# Autodesk Inventor assembly: chwytak
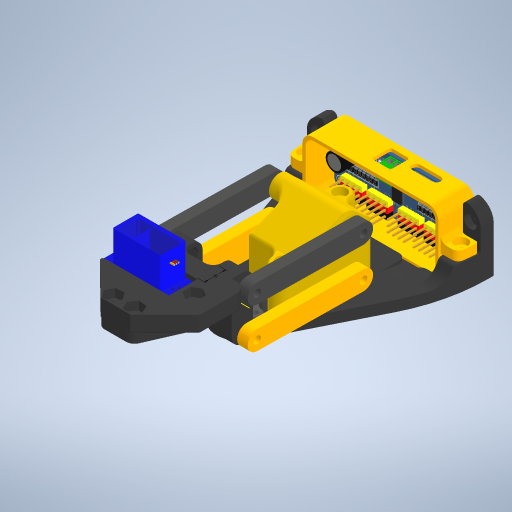
[picture p0: Inventor's stored thumbnail of the model, 512x512]
Saved by Autodesk Inventor 2023 (Build 270158000, 158)
## iProperties
Created: 2024-05-12
Part Number: chwytak
Document SubType Name: Assembly
Designer: kamil
Author: kamil
## Documents named in this file (12)
- C:\Users\kamil\Documents\PROJECTS - repos\ModBot---Projekt-Zespolowy\mechanics\modul_chwytaka\chwytak.iam
- C:\Users\kamil\Documents\PROJECTS - repos\ModBot---Projekt-Zespolowy\mechanics\modul_chwytaka\belka.ipt
- C:\Users\kamil\Documents\PROJECTS - repos\ModBot---Projekt-Zespolowy\mechanics\modul_chwytaka\Towerpro Micro Servo 9g.ipt
- C:\Users\kamil\Documents\PROJECTS - repos\ModBot---Projekt-Zespolowy\mechanics\modul_chwytaka\A1.ipt
- C:\Users\kamil\Documents\PROJECTS - repos\ModBot---Projekt-Zespolowy\mechanics\modul_chwytaka\uchwyt_serwa.ipt
- C:\Users\kamil\Documents\PROJECTS - repos\ModBot---Projekt-Zespolowy\mechanics\modul_chwytaka\belka_2.ipt
- C:\Users\kamil\Documents\PROJECTS - repos\ModBot---Projekt-Zespolowy\mechanics\modul_chwytaka\uchwyt_gorny.ipt
- C:\Users\kamil\Documents\PROJECTS - repos\ModBot---Projekt-Zespolowy\mechanics\STEP\pca9685.ipt
- C:\Users\kamil\Documents\PROJECTS - repos\ModBot---Projekt-Zespolowy\mechanics\chwytak_mocowanie.ipt
- C:\Users\kamil\Documents\PROJECTS - repos\ModBot---Projekt-Zespolowy\mechanics\STEP\Pololu Ball Caster with 3_8_ Metal Ball.ipt
- C:\Users\kamil\Documents\PROJECTS - repos\ModBot---Projekt-Zespolowy\mechanics\pca_obudowa.iam
- C:\Users\kamil\Documents\PROJECTS - repos\ModBot---Projekt-Zespolowy\mechanics\modul_chwytaka\chwytak_montaz.ipt
## Components (15 placed, 11 different names)
1. belka:1 — Zestawiające:4, Zestawiające:5, Kątowe:1, Zestawiające:12, Równoległe:3, Równoległe:6, Zestawiające:46
2. Towerpro Micro Servo 9g:1 — Zestawiające:1, Zestawiające:2, Równoległe:1, Zestawiające:3, Zestawiające:6, Zestawiające:7, Zestawiające:8, Zestawiające:9
3. A1:1 — Zestawiające:2, Zestawiające:3, Zestawiające:4, Zestawiające:5, Kątowe:1
4. uchwyt_serwa:1 — Zestawiające:7, Zestawiające:8, Zestawiające:9, Zestawiające:10, Zestawiające:11, Zestawiające:13, Zestawiające:14, Zestawiające:37, Zestawiające:40
5. belka_2:1 — Zestawiające:10, Zestawiające:11, Zestawiające:12, Równoległe:2, Kątowe:2
6. uchwyt_gorny:1 — Zestawiające:13, Zestawiające:14, Zestawiające:38, Zestawiające:39
7. belka_2:2 — Równoległe:2, Kątowe:2, Równoległe:4, Zestawiające:39
8. belka_2:3 — Równoległe:3, Równoległe:4, Zestawiające:38, Zestawiające:47, Zestawiające:48
9. chwytak_mocowanie:1 — Zestawiające:35, Zestawiające:36, Zestawiające:37, Równoległe:5, Równoległe:6, Zestawiające:40, Zestawiające:41, Zestawiające:42, Zestawiające:43, Zestawiające:44, Równoległe:7, Równoległe:8, Zestawiające:45, Równoległe:9
10. Pololu Ball Caster with 3_8_ Metal Ball:1 — Zestawiające:41, Zestawiające:42, Zestawiające:43, Zestawiające:44
11. pca9685:1 — Zestawiające:35, Zestawiające:36, Równoległe:5
12. pca_obudowa:1 [sub-assembly] — Równoległe:7, Równoległe:8, Zestawiające:45, Równoległe:9, Zestawiające:52, Zestawiające:53, Zestawiające:54
13. chwytak_montaz:1 — Zestawiające:46, Zestawiające:47, Zestawiające:48, Zestawiające:49, Kątowe:3, Zestawiające:50, Zestawiające:51
14. Towerpro Micro Servo 9g:2 — Zestawiające:49, Kątowe:3, Zestawiające:50, Zestawiające:51
15. pca9685:2 — Zestawiające:52, Zestawiające:53, Zestawiające:54
## Relationships (46: Mate 34, Flush 9, Angle 3)
- Zestawiające:1 [Mate]: Towerpro Micro Servo 9g:1
- Zestawiające:2 [Mate]: Towerpro Micro Servo 9g:1 ↔ A1:1
- Równoległe:1 [Flush]: Towerpro Micro Servo 9g:1
- Zestawiające:3 [Mate]: Towerpro Micro Servo 9g:1 ↔ A1:1
- Zestawiające:4 [Mate]: belka:1 ↔ A1:1
- Zestawiające:5 [Mate]: belka:1 ↔ A1:1
- Kątowe:1 [Angle] (180 deg): belka:1 ↔ A1:1
- Zestawiające:6 [Mate]: Towerpro Micro Servo 9g:1
- Zestawiające:7 [Mate]: Towerpro Micro Servo 9g:1 ↔ uchwyt_serwa:1
- Zestawiające:8 [Mate] (0.5 mm): Towerpro Micro Servo 9g:1 ↔ uchwyt_serwa:1
- Zestawiające:9 [Mate]: Towerpro Micro Servo 9g:1 ↔ uchwyt_serwa:1
- Zestawiające:10 [Mate] (2 mm): uchwyt_serwa:1 ↔ belka_2:1
- Zestawiające:11 [Mate]: uchwyt_serwa:1 ↔ belka_2:1
- Zestawiające:12 [Mate]: belka:1 ↔ belka_2:1
- Zestawiające:13 [Mate]: uchwyt_serwa:1 ↔ uchwyt_gorny:1
- Zestawiające:14 [Mate]: uchwyt_serwa:1 ↔ uchwyt_gorny:1
- Równoległe:2 [Flush]: belka_2:1 ↔ belka_2:2
- Kątowe:2 [Angle] (180 deg): belka_2:1 ↔ belka_2:2
- Równoległe:3 [Flush]: belka:1 ↔ belka_2:3
- Równoległe:4 [Flush]: belka_2:2 ↔ belka_2:3
- Zestawiające:35 [Mate] (2 mm): chwytak_mocowanie:1 ↔ pca9685:1
- Zestawiające:36 [Mate] (2 mm): chwytak_mocowanie:1 ↔ pca9685:1
- Zestawiające:37 [Mate]: uchwyt_serwa:1 ↔ chwytak_mocowanie:1
- Równoległe:5 [Flush] (-11 mm): chwytak_mocowanie:1 ↔ pca9685:1
- Zestawiające:38 [Mate]: uchwyt_gorny:1 ↔ belka_2:3
- Zestawiające:39 [Mate]: uchwyt_gorny:1 ↔ belka_2:2
- Równoległe:6 [Flush] (17.75 mm): belka:1 ↔ chwytak_mocowanie:1
- Zestawiające:40 [Mate] (25 mm): uchwyt_serwa:1 ↔ chwytak_mocowanie:1
- Zestawiające:41 [Mate] (-7 mm): chwytak_mocowanie:1 ↔ Pololu Ball Caster with 3_8_ Metal Ball:1
- Zestawiające:42 [Mate] (-41 mm): chwytak_mocowanie:1 ↔ Pololu Ball Caster with 3_8_ Metal Ball:1
- Zestawiające:43 [Mate] (72 mm): chwytak_mocowanie:1 ↔ Pololu Ball Caster with 3_8_ Metal Ball:1
- Zestawiające:44 [Mate] (72 mm): chwytak_mocowanie:1 ↔ Pololu Ball Caster with 3_8_ Metal Ball:1
- Równoległe:7 [Flush]: chwytak_mocowanie:1 ↔ pca_obudowa:1
- Równoległe:8 [Flush] (-9 mm): chwytak_mocowanie:1 ↔ pca_obudowa:1
- Zestawiające:45 [Mate]: chwytak_mocowanie:1 ↔ pca_obudowa:1
- Równoległe:9 [Flush]: chwytak_mocowanie:1 ↔ pca_obudowa:1
- Zestawiające:46 [Mate]: belka:1 ↔ chwytak_montaz:1
- Zestawiające:47 [Mate]: belka_2:3 ↔ chwytak_montaz:1
- Zestawiające:48 [Mate] (2 mm): belka_2:3 ↔ chwytak_montaz:1
- Zestawiające:49 [Mate]: chwytak_montaz:1 ↔ Towerpro Micro Servo 9g:2
- Kątowe:3 [Angle] (0 deg): chwytak_montaz:1 ↔ Towerpro Micro Servo 9g:2
- Zestawiające:50 [Mate]: chwytak_montaz:1 ↔ Towerpro Micro Servo 9g:2
- Zestawiające:51 [Mate] (0.5 mm): chwytak_montaz:1 ↔ Towerpro Micro Servo 9g:2
- Zestawiające:52 [Mate]: pca_obudowa:1 ↔ pca9685:2
- Zestawiające:53 [Mate]: pca_obudowa:1 ↔ pca9685:2
- Zestawiające:54 [Mate]: pca_obudowa:1 ↔ pca9685:2
